# Autodesk Inventor assembly: Sensor_Halterung_Klemme
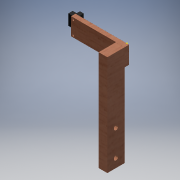
[picture p0: Inventor's stored thumbnail of the model, 180x180]
Saved by Autodesk Inventor 2018 (Build 220112000, 112)
## iProperties
Created: 2018-03-26
Part Number: Sensor_Halterung_Klemme
Material: Generisch
Document SubType Name: Assembly
Designer: Julian
Author: Julian
## Documents named in this file (4)
- C:\Users\Julian\Desktop\Schule\5AHME\Diplomarbeit\Git\fuettr_prototype\Mechanical\Inventorskizzen\Sensor_Halterung_Klemme.iam
- C:\Users\Julian\Desktop\Schule\5AHME\Diplomarbeit\Git\fuettr_prototype\Mechanical\Inventorskizzen\OPB732.ipt
- C:\Users\Julian\Desktop\Schule\5AHME\Diplomarbeit\Git\fuettr_prototype\Mechanical\Inventorskizzen\Sensor_Halterung_Teil1.ipt
- C:\Users\Julian\Desktop\Schule\5AHME\Diplomarbeit\Git\fuettr_prototype\Mechanical\Inventorskizzen\Sensor_Halterung_Teil2ipt.ipt
## Components (3 placed, 3 different names)
1. OPB732:1 — Starr:2
2. Sensor_Halterung_Teil1:1 — Starr:1
3. Sensor_Halterung_Teil2ipt:1 — Starr:1, Starr:2
## Relationships (2: WeldJoint 2)
- Starr:1 [WeldJoint]: Sensor_Halterung_Teil1:1 ↔ Sensor_Halterung_Teil2ipt:1
- Starr:2 [WeldJoint]: OPB732:1 ↔ Sensor_Halterung_Teil2ipt:1
